# Autodesk Inventor assembly: synth-screw-mount
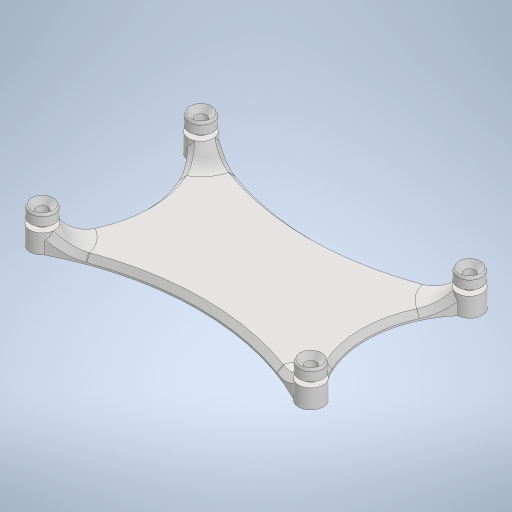
[picture p0: Inventor's stored thumbnail of the model, 512x512]
Saved by Autodesk Inventor 2024.1 (Build 281209000, 209)
## iProperties
Created: 2025-04-08
Part Number: synth-screw-mount
Document SubType Name: Assembly
Designer: iwheard
Author: iwheard
## Documents named in this file (4)
- C:\Users\iwheard\Documents\0004-CAD\3D-cad-main\low-poly-audio\synth-mount\synth-screw-mount.iam
- C:\Users\iwheard\Documents\0000-kicad\projects\personal-projects\diode-ladder-filter-synth-module\diode-ladder-filter-synth-module\diode-ladder-filter-synth-module.iam
- C:\Users\iwheard\Documents\0004-CAD\3D-cad-main\low-poly-audio\synth-mount\synth-mounting.ipt
- C:\Users\iwheard\Documents\0004-CAD\3D-cad-main\low-poly-audio\synth-mount\screw-holders.ipt
## Components (3 placed, 3 different names)
1. diode-ladder-filter-synth-module:1 [sub-assembly] — Flush:1, Flush:2, Flush:3, Flush:4
2. synth-mounting:1 — Flush:1, Flush:2
3. screw-holders:1 — Flush:3, Flush:4
## Relationships (4: Flush 4)
- Flush:1: diode-ladder-filter-synth-module:1 ↔ synth-mounting:1
- Flush:2: diode-ladder-filter-synth-module:1 ↔ synth-mounting:1
- Flush:3: diode-ladder-filter-synth-module:1 ↔ screw-holders:1
- Flush:4: diode-ladder-filter-synth-module:1 ↔ screw-holders:1
